# Autodesk Inventor assembly: nc_nhk23
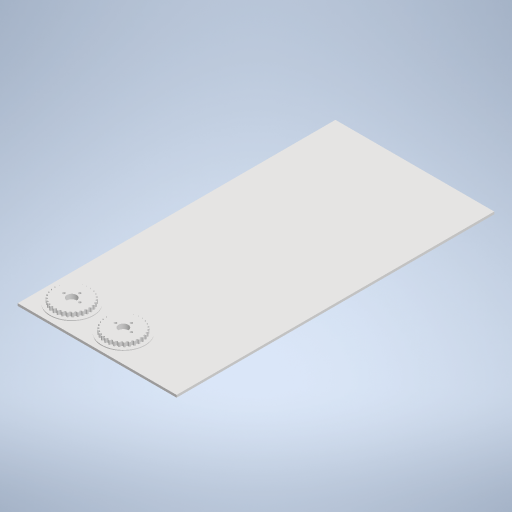
[picture p0: Inventor's stored thumbnail of the model, 512x512]
Saved by Autodesk Inventor 2023 (Build 270158000, 158)
## iProperties
Created: 2022-04-30
Part Number: nc_nhk23
Document SubType Name: Assembly
Designer: yuta
Author: yuta
## Documents named in this file (3)
- C:\Users\yuta\Documents\NHK\nc_nhk23.iam
- C:\Users\yuta\Documents\NHK\NC.port.ipt
- C:\Users\yuta\Documents\NHK\射出_プーリ30.ipt
## Components (3 placed, 2 different names)
1. NC.port:1 — メイト:1, メイト:2, メイト:3, メイト:4, メイト:5
2. 射出_プーリ30:1 — メイト:1, メイト:2, メイト:3, メイト:6
3. 射出_プーリ30:2 — メイト:4, メイト:5, メイト:6
## Relationships (6: Mate 6)
- メイト:1 [Mate]: NC.port:1 ↔ 射出_プーリ30:1
- メイト:2 [Mate] (-34 mm): NC.port:1 ↔ 射出_プーリ30:1
- メイト:3 [Mate] (-34 mm): NC.port:1 ↔ 射出_プーリ30:1
- メイト:4 [Mate]: NC.port:1 ↔ 射出_プーリ30:2
- メイト:5 [Mate] (-34 mm): NC.port:1 ↔ 射出_プーリ30:2
- メイト:6 [Mate] (65 mm): 射出_プーリ30:1 ↔ 射出_プーリ30:2
